# Autodesk Inventor assembly: main2
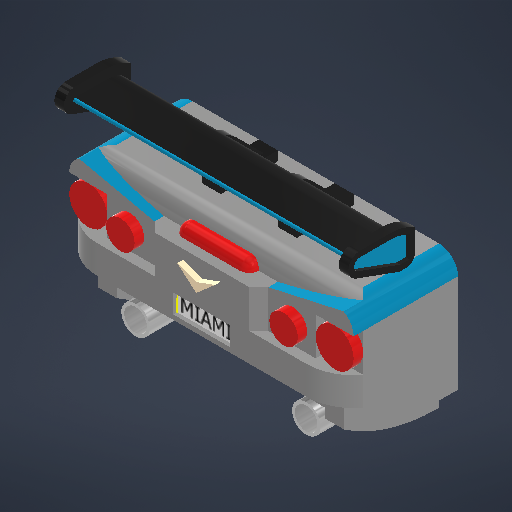
[picture p0: Inventor's stored thumbnail of the model, 512x512]
Saved by Autodesk Inventor 2026.2 (Build 302298000, 298)
## iProperties
Created: 2026-08-18
Part Number: main2
Document SubType Name: Assembly
Designer: wojsl
Author: wojsl
## Documents named in this file (3)
- C:\Users\wojsl\OneDrive\Pulpit\cad\samochód\main2.iam
- C:\Users\wojsl\OneDrive\Pulpit\cad\samochód\spoiler.ipt
- C:\Users\wojsl\OneDrive\Pulpit\cad\samochód\zderzak.ipt
## Components (2 placed, 2 different names)
1. spoiler:1 — Wstawiające:1
2. zderzak:1 — Wstawiające:1
## Relationships (1: Insert 1)
- Wstawiające:1 [Insert]: spoiler:1 ↔ zderzak:1
